# Autodesk Inventor assembly: cupula_partes
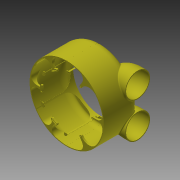
[picture p0: Inventor's stored thumbnail of the model, 180x180]
Saved by Autodesk Inventor 2015 (Build 190159000, 159)
## iProperties
Created: 2015-06-04
Part Number: cupula_partes
Document SubType Name: Assembly
Designer: david_000
Author: david_000
## Documents named in this file (4)
- C:\Users\david_000\Desktop\minibot-code\mechanics\cupula_partes.iam
- C:\Users\david_000\Desktop\minibot-code\mechanics\cupula2_parte_trasera.ipt
- C:\Users\david_000\Desktop\minibot-code\mechanics\cupula2_parte_delantera.ipt
- C:\Users\david_000\Desktop\minibot-code\mechanics\cupula2_parte_delantera_2.ipt
## Components (5 placed, 3 different names)
1. cupula2_parte_delantera:1 — Coincidencia:1, Coincidencia:2, Nivelación:1
2. cupula2_parte_delantera_2:1 — Coincidencia:1, Coincidencia:2, Nivelación:1, Coincidencia:7, Nivelación:4, Coincidencia:8
3. cupula2_parte_trasera:1 — Coincidencia:3, Coincidencia:5, Coincidencia:6, Nivelación:2, Nivelación:3, Coincidencia:7, Nivelación:4
4. cupula2_parte_trasera:2 — Coincidencia:3, Coincidencia:4, Coincidencia:5, Nivelación:3, Coincidencia:8
5. cupula2_parte_trasera:3 — Coincidencia:4, Coincidencia:6, Nivelación:2
## Relationships (12: Mate 8, Flush 4)
- Coincidencia:1 [Mate]: cupula2_parte_delantera:1 ↔ cupula2_parte_delantera_2:1
- Coincidencia:2 [Mate]: cupula2_parte_delantera:1 ↔ cupula2_parte_delantera_2:1
- Nivelación:1 [Flush]: cupula2_parte_delantera:1 ↔ cupula2_parte_delantera_2:1
- Coincidencia:3 [Mate]: cupula2_parte_trasera:1 ↔ cupula2_parte_trasera:2
- Coincidencia:4 [Mate]: cupula2_parte_trasera:2 ↔ cupula2_parte_trasera:3
- Coincidencia:5 [Mate]: cupula2_parte_trasera:1 ↔ cupula2_parte_trasera:2
- Coincidencia:6 [Mate]: cupula2_parte_trasera:1 ↔ cupula2_parte_trasera:3
- Nivelación:2 [Flush]: cupula2_parte_trasera:1 ↔ cupula2_parte_trasera:3
- Nivelación:3 [Flush]: cupula2_parte_trasera:1 ↔ cupula2_parte_trasera:2
- Coincidencia:7 [Mate]: cupula2_parte_delantera_2:1 ↔ cupula2_parte_trasera:1
- Nivelación:4 [Flush]: cupula2_parte_delantera_2:1 ↔ cupula2_parte_trasera:1
- Coincidencia:8 [Mate]: cupula2_parte_delantera_2:1 ↔ cupula2_parte_trasera:2
